# Autodesk Inventor assembly: main_pcb.brd
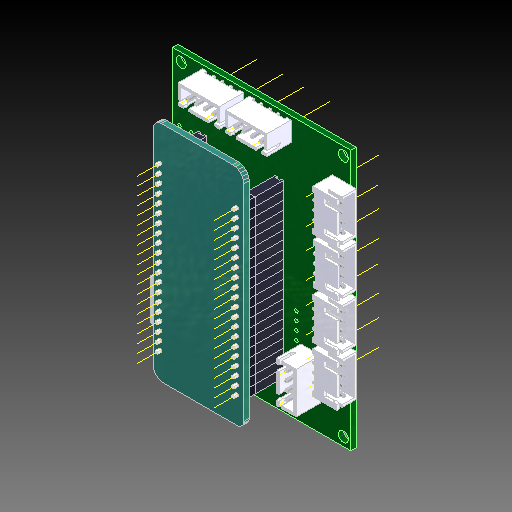
[picture p0: Inventor's stored thumbnail of the model, 512x512]
Saved by Autodesk Inventor 2020 (Build 240168000, 168)
## iProperties
Created: 2021-08-05
Part Number: main_pcb.brd
Document SubType Name: Assembly
Designer: Петров Иван
Mass: 18.6028 g
Surface Area: 275.031 cm^2
Volume: 13.5279 cm^3
Density: 1.37514 g/cm^3
Author: Петров Иван
## Documents named in this file (7)
- E:\IVAN\Ivan_desktop\Kvantorium\Projects\RoboPatrol\electronic\MAIN_PCB\main_pcb.brd.iam
- E:\IVAN\Ivan_desktop\Kvantorium\Projects\RoboPatrol\design\standart_components\PBS-1.ipt
- E:\IVAN\Ivan_desktop\Kvantorium\Projects\RoboPatrol\design\standart_components\connectrs\JST - XH - Thru (R) - 4Pin - 2.54mm.ipt
- E:\IVAN\Ivan_desktop\Kvantorium\Projects\RoboPatrol\design\standart_components\connectrs\JST - XH - Thru (V) - 4Pin - 2.54mm.ipt
- E:\IVAN\Ivan_desktop\Kvantorium\Projects\RoboPatrol\electronic\MAIN_PCB\main_pcb.brd.ipt
- E:\IVAN\Ivan_desktop\Kvantorium\Projects\RoboPatrol\design\standart_components\CONN HEADER VERT 1POS 2.54MM.ipt
- E:\IVAN\Ivan_desktop\Kvantorium\Projects\RoboPatrol\electronic\MAIN_PCB\opencm904.ipt
## Components (91 placed, 6 different names)
1. main_pcb.brd:1 — Совмещение:15, Совмещение:16, Совмещение:17, Совмещение:18, Совмещение:19, Совмещение:20, Совмещение:26, Совмещение:27, Совмещение:28, Совмещение:29, Совмещение:30, Совмещение:31
2. PBS-1:1
3. JST - XH - Thru (R) - 4Pin - 2.54mm:1
4. JST - XH - Thru (R) - 4Pin - 2.54mm:2
5. JST - XH - Thru (V) - 4Pin - 2.54mm:1
6. JST - XH - Thru (V) - 4Pin - 2.54mm:2
7. JST - XH - Thru (R) - 4Pin - 2.54mm:3 — Совмещение:18, Совмещение:19, Совмещение:20
8. JST - XH - Thru (R) - 4Pin - 2.54mm:4 — Совмещение:15, Совмещение:16, Совмещение:17
9. untitled.brdКонтур:1 — Совмещение:23, Совмещение:24, Совмещение:25
10. JST - XH - Thru (V) - 4Pin - 2.54mm:3 — Совмещение:26, Совмещение:27, Совмещение:28
11. JST - XH - Thru (V) - 4Pin - 2.54mm:4 — Совмещение:29, Совмещение:30, Совмещение:31
12. PBS-1:2 — Совмещение:21, Совмещение:22, Заподлицо:1
13. PBS-1:3
14. PBS-1:4
15. PBS-1:5
16. PBS-1:6
17. PBS-1:7
18. PBS-1:8
19. PBS-1:9
20. PBS-1:10
21. PBS-1:11
22. PBS-1:12
23. PBS-1:13
24. PBS-1:14
25. PBS-1:15
26. PBS-1:16
27. PBS-1:17
28. PBS-1:18
29. PBS-1:19
30. PBS-1:20
31. PBS-1:21
32. PBS-1:22
33. PBS-1:23
34. PBS-1:24
35. PBS-1:25
36. PBS-1:26
37. PBS-1:27
38. PBS-1:28
39. PBS-1:29
40. PBS-1:30
41. PBS-1:31
42. PBS-1:32
43. PBS-1:33
44. PBS-1:34
45. PBS-1:35
46. PBS-1:36
47. PBS-1:37
48. PBS-1:38
49. PBS-1:39
50. PBS-1:40
51. PBS-1:41
52. CONN HEADER VERT 1POS 2.54MM:1 — Совмещение:21, Совмещение:22, Заподлицо:1, Совмещение:23, Совмещение:24
53. CONN HEADER VERT 1POS 2.54MM:2
54. CONN HEADER VERT 1POS 2.54MM:3
55. CONN HEADER VERT 1POS 2.54MM:4
56. CONN HEADER VERT 1POS 2.54MM:5
57. CONN HEADER VERT 1POS 2.54MM:6
58. CONN HEADER VERT 1POS 2.54MM:7
59. CONN HEADER VERT 1POS 2.54MM:8
60. CONN HEADER VERT 1POS 2.54MM:9
61. CONN HEADER VERT 1POS 2.54MM:10
62. CONN HEADER VERT 1POS 2.54MM:11
63. CONN HEADER VERT 1POS 2.54MM:12
64. CONN HEADER VERT 1POS 2.54MM:13
65. CONN HEADER VERT 1POS 2.54MM:14
66. CONN HEADER VERT 1POS 2.54MM:15
67. CONN HEADER VERT 1POS 2.54MM:16
68. CONN HEADER VERT 1POS 2.54MM:17
69. CONN HEADER VERT 1POS 2.54MM:18
70. CONN HEADER VERT 1POS 2.54MM:19
71. CONN HEADER VERT 1POS 2.54MM:20
72. CONN HEADER VERT 1POS 2.54MM:21
73. CONN HEADER VERT 1POS 2.54MM:22
74. CONN HEADER VERT 1POS 2.54MM:23
75. CONN HEADER VERT 1POS 2.54MM:24
76. CONN HEADER VERT 1POS 2.54MM:25
77. CONN HEADER VERT 1POS 2.54MM:26
78. CONN HEADER VERT 1POS 2.54MM:27
79. CONN HEADER VERT 1POS 2.54MM:28
80. CONN HEADER VERT 1POS 2.54MM:29
81. CONN HEADER VERT 1POS 2.54MM:30
82. CONN HEADER VERT 1POS 2.54MM:31
83. CONN HEADER VERT 1POS 2.54MM:32
84. CONN HEADER VERT 1POS 2.54MM:33
85. CONN HEADER VERT 1POS 2.54MM:34
86. CONN HEADER VERT 1POS 2.54MM:35
87. CONN HEADER VERT 1POS 2.54MM:36
88. CONN HEADER VERT 1POS 2.54MM:37
89. CONN HEADER VERT 1POS 2.54MM:38
90. CONN HEADER VERT 1POS 2.54MM:39
91. CONN HEADER VERT 1POS 2.54MM:40 — Совмещение:25
## Component patterns: (40 elements, first: PBS-1:2), (40 elements, first: CONN HEADER VERT 1POS 2.54MM:1)
## Relationships (33: Mate 31, Angle 1, Flush 1)
- [Mate]: main_pcb.brd:1 ↔ PBS-1:2
- [Angle] (90 deg): main_pcb.brd:1 ↔ PBS-1:2
- [Mate]: main_pcb.brd:1 ↔ PBS-1:2
- [Mate]: main_pcb.brd:1 ↔ JST - XH - Thru (R) - 4Pin - 2.54mm:1
- [Mate]: main_pcb.brd:1 ↔ JST - XH - Thru (R) - 4Pin - 2.54mm:1
- [Mate]: main_pcb.brd:1 ↔ JST - XH - Thru (R) - 4Pin - 2.54mm:1
- [Mate]: main_pcb.brd:1 ↔ JST - XH - Thru (R) - 4Pin - 2.54mm:2
- [Mate]: main_pcb.brd:1 ↔ JST - XH - Thru (R) - 4Pin - 2.54mm:2
- [Mate]: main_pcb.brd:1 ↔ JST - XH - Thru (R) - 4Pin - 2.54mm:2
- [Mate]: main_pcb.brd:1 ↔ JST - XH - Thru (V) - 4Pin - 2.54mm:1
- [Mate]: main_pcb.brd:1 ↔ JST - XH - Thru (V) - 4Pin - 2.54mm:1
- [Mate]: main_pcb.brd:1 ↔ JST - XH - Thru (V) - 4Pin - 2.54mm:1
- [Mate]: main_pcb.brd:1 ↔ JST - XH - Thru (V) - 4Pin - 2.54mm:2
- [Mate]: main_pcb.brd:1 ↔ JST - XH - Thru (V) - 4Pin - 2.54mm:2
- [Mate]: main_pcb.brd:1 ↔ JST - XH - Thru (V) - 4Pin - 2.54mm:2
- Совмещение:15 [Mate]: main_pcb.brd:1 ↔ JST - XH - Thru (R) - 4Pin - 2.54mm:4
- Совмещение:16 [Mate]: main_pcb.brd:1 ↔ JST - XH - Thru (R) - 4Pin - 2.54mm:4
- Совмещение:17 [Mate]: main_pcb.brd:1 ↔ JST - XH - Thru (R) - 4Pin - 2.54mm:4
- Совмещение:18 [Mate]: main_pcb.brd:1 ↔ JST - XH - Thru (R) - 4Pin - 2.54mm:3
- Совмещение:19 [Mate]: main_pcb.brd:1 ↔ JST - XH - Thru (R) - 4Pin - 2.54mm:3
- Совмещение:20 [Mate]: main_pcb.brd:1 ↔ JST - XH - Thru (R) - 4Pin - 2.54mm:3
- Совмещение:21 [Mate]: PBS-1:2 ↔ CONN HEADER VERT 1POS 2.54MM:1
- Совмещение:22 [Mate]: PBS-1:2 ↔ CONN HEADER VERT 1POS 2.54MM:1
- Заподлицо:1 [Flush]: PBS-1:2 ↔ CONN HEADER VERT 1POS 2.54MM:1
- Совмещение:23 [Mate]: untitled.brdКонтур:1 ↔ CONN HEADER VERT 1POS 2.54MM:1
- Совмещение:24 [Mate]: untitled.brdКонтур:1 ↔ CONN HEADER VERT 1POS 2.54MM:1
- Совмещение:25 [Mate]: untitled.brdКонтур:1 ↔ CONN HEADER VERT 1POS 2.54MM:40
- Совмещение:26 [Mate]: main_pcb.brd:1 ↔ JST - XH - Thru (V) - 4Pin - 2.54mm:3
- Совмещение:27 [Mate]: main_pcb.brd:1 ↔ JST - XH - Thru (V) - 4Pin - 2.54mm:3
- Совмещение:28 [Mate]: main_pcb.brd:1 ↔ JST - XH - Thru (V) - 4Pin - 2.54mm:3
- Совмещение:29 [Mate]: main_pcb.brd:1 ↔ JST - XH - Thru (V) - 4Pin - 2.54mm:4
- Совмещение:30 [Mate]: main_pcb.brd:1 ↔ JST - XH - Thru (V) - 4Pin - 2.54mm:4
- Совмещение:31 [Mate]: main_pcb.brd:1 ↔ JST - XH - Thru (V) - 4Pin - 2.54mm:4
